# Autodesk Inventor assembly: link_arm1_5
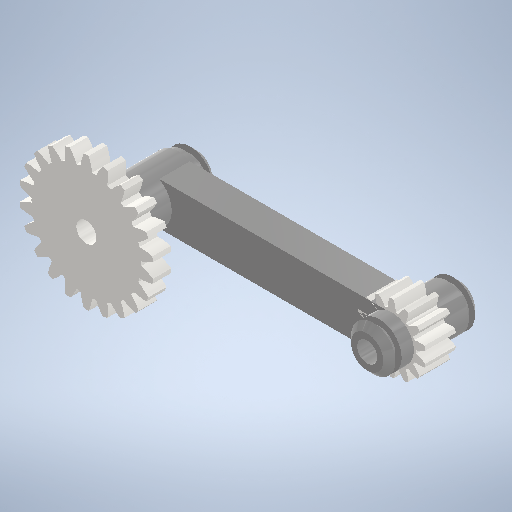
[picture p0: Inventor's stored thumbnail of the model, 512x512]
Saved by Autodesk Inventor 2025 (Build 290162000, 162)
## iProperties
Created: 2025-10-23
Part Number: link_arm1_5
Document SubType Name: Assembly
Designer: sooo1
Author: sooo1
## Documents named in this file (7)
- C:\Users\sooo1\Documents\Inventor\MOBITOUCH\final\stroke_module_1\link_arm1_5.iam
- C:\Users\sooo1\Documents\Inventor\MOBITOUCH\final\stroke_module_1\link_arm_1_5.ipt
- C:\Users\sooo1\Documents\Inventor\MOBITOUCH\final\stroke_module_1\link_arm1_5\デザイン アクセラレータ\平歯車2.iam
- C:\Users\sooo1\Documents\Inventor\MOBITOUCH\final\stroke_module_1\spacer_Φ3.2_4.ipt
- C:\Users\sooo1\Documents\Inventor\MOBITOUCH\final\stroke_module_1\spacer_Φ3.2_6.ipt
- C:\Users\sooo1\Documents\Inventor\MOBITOUCH\final\stroke_module_1\spacer_Φ3.2_5.ipt
- C:\Users\sooo1\Documents\Inventor\MOBITOUCH\final\stroke_module_1\平歯車1.iam
## Components (6 placed, 5 different names)
1. link_arm_1_5:1 — フラッシュ:1, フラッシュ:2, フラッシュ:3, メイト:2, メイト:3, メイト:8, メイト:9, メイト:10, メイト:11, メイト:12, メイト:13, メイト:14, 角度:2, フラッシュ:4
2. 平歯車:1 [sub-assembly] — メイト:2, メイト:3, 角度:1
3. spacer_Φ3.2_6:1 — メイト:8, メイト:9
4. spacer_Φ3.2_5:1 — メイト:10, メイト:11
5. spacer_Φ3.2_4:1 — メイト:12, メイト:13
6. 平歯車:2 [sub-assembly] — メイト:14, 角度:2, フラッシュ:4
## Relationships (15: Mate 9, Flush 4, Angle 2)
- フラッシュ:1 [Flush]: link_arm_1_5:1
- フラッシュ:2 [Flush]: link_arm_1_5:1
- フラッシュ:3 [Flush]: link_arm_1_5:1
- メイト:2 [Mate]: link_arm_1_5:1 ↔ 平歯車:1
- メイト:3 [Mate]: link_arm_1_5:1 ↔ 平歯車:1
- 角度:1 [Angle] (90 deg): 平歯車:1
- メイト:8 [Mate]: link_arm_1_5:1 ↔ spacer_Φ3.2_6:1
- メイト:9 [Mate]: link_arm_1_5:1 ↔ spacer_Φ3.2_6:1
- メイト:10 [Mate]: link_arm_1_5:1 ↔ spacer_Φ3.2_5:1
- メイト:11 [Mate]: link_arm_1_5:1 ↔ spacer_Φ3.2_5:1
- メイト:12 [Mate]: link_arm_1_5:1 ↔ spacer_Φ3.2_4:1
- メイト:13 [Mate]: link_arm_1_5:1 ↔ spacer_Φ3.2_4:1
- メイト:14 [Mate]: link_arm_1_5:1 ↔ 平歯車:2
- 角度:2 [Angle] (0 deg): link_arm_1_5:1 ↔ 平歯車:2
- フラッシュ:4 [Flush]: link_arm_1_5:1 ↔ 平歯車:2
